# Autodesk Inventor assembly: AS_Мехатрон R1
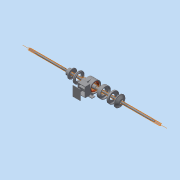
[picture p0: Inventor's stored thumbnail of the model, 180x180]
Saved by Autodesk Inventor 2016 SP1 (Build 200210100, 210)
## iProperties
Created: 2016-04-25
Part Number: AS_Мехатрон R1
Material: Типовые
Document SubType Name: Assembly
Designer: AS
Author: AS
## Documents named in this file (9)
- D:\D_мои документы\Алексей\Мехатрон\AS_Мехатрон R1.iam
- D:\D_мои документы\Алексей\Мехатрон\Vint.ipt
- D:\D_мои документы\Алексей\Мехатрон\2 крышка.ipt
- D:\D_мои документы\Алексей\Мехатрон\Деталь 3.ipt
- D:\D_мои документы\Алексей\Мехатрон\Деталь 4.ipt
- D:\D_мои документы\Алексей\Мехатрон\Деталь 5.ipt
- D:\D_мои документы\Алексей\Мехатрон\Деталь 6.ipt
- D:\D_мои документы\Алексей\Мехатрон\Полый вал.iam
- D:\D_мои документы\Алексей\Мехатрон\Корпус 1 сборка.iam
## Components (8 placed, 8 different names)
1. Vint:1 — Совмещение:1
2. 2 крышка:1 — Заподлицо:2, Совмещение:3
3. Деталь 3:1 — Заподлицо:4, Совмещение:4
4. Деталь 4:1 — Заподлицо:5, Совмещение:5, Совмещение:7
5. Деталь 5:1 — Заподлицо:6, Совмещение:6
6. Деталь 6:1 — Заподлицо:7, Совмещение:7
7. Полый вал:1 [sub-assembly] — Совмещение:9
8. Корпус 1 сборка:1 [sub-assembly] — Совмещение:10, Заподлицо:8, Заподлицо:9
## Relationships (15: Mate 8, Flush 7)
- Совмещение:1 [Mate]: Vint:1
- Заподлицо:2 [Flush]: 2 крышка:1
- Совмещение:3 [Mate]: 2 крышка:1
- Заподлицо:4 [Flush]: Деталь 3:1
- Совмещение:4 [Mate]: Деталь 3:1
- Заподлицо:5 [Flush]: Деталь 4:1
- Совмещение:5 [Mate]: Деталь 4:1
- Заподлицо:6 [Flush]: Деталь 5:1
- Совмещение:6 [Mate]: Деталь 5:1
- Заподлицо:7 [Flush]: Деталь 6:1
- Совмещение:7 [Mate]: Деталь 4:1 ↔ Деталь 6:1
- Совмещение:9 [Mate]: Полый вал:1
- Совмещение:10 [Mate]: Корпус 1 сборка:1
- Заподлицо:8 [Flush]: Корпус 1 сборка:1
- Заподлицо:9 [Flush]: Корпус 1 сборка:1
